# Autodesk Inventor assembly: marco
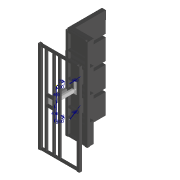
[picture p0: Inventor's stored thumbnail of the model, 180x180]
Saved by Autodesk Inventor 2021 (Build 250183000, 183)
## iProperties
Created: 2021-04-11
Part Number: marco
Document SubType Name: Assembly
Designer: equip
Mass: 525959 g
Surface Area: 133006 cm^2
Volume: 315655 cm^3
Density: 1.66625 g/cm^3
_SolveAssemblyDoc: Frame Generator Solve Assembly
_Version: 25.0.0
Author: equip
## Documents named in this file (12)
- C:\Users\Santiago Suárez\Documents\GitHub\Dis.-Mecatronico-E6\inventor proyecto\marco.iam
- C:\Users\Santiago Suárez\Documents\GitHub\Dis.-Mecatronico-E6\inventor proyecto\placa centro.ipt
- C:\Users\Santiago Suárez\Documents\GitHub\Dis.-Mecatronico-E6\inventor proyecto\Silla del marco.ipt
- C:\Users\Santiago Suárez\Documents\GitHub\Dis.-Mecatronico-E6\inventor proyecto\cilindro\cilindro.iam
- C:\Users\Santiago Suárez\Documents\GitHub\Dis.-Mecatronico-E6\inventor proyecto\marco inferior.ipt
- C:\Users\Santiago Suárez\Documents\GitHub\Dis.-Mecatronico-E6\inventor proyecto\marco\Frame\Marco Inferior.iam
- C:\Users\Santiago Suárez\Documents\GitHub\Dis.-Mecatronico-E6\inventor proyecto\MarcoSuperior.iam
- C:\Users\Santiago Suárez\Documents\GitHub\Dis.-Mecatronico-E6\inventor proyecto\Motor1.ipt
- C:\Users\Santiago Suárez\Documents\GitHub\Dis.-Mecatronico-E6\inventor proyecto\PlacaInferior.ipt
- C:\Users\Santiago Suárez\Documents\GitHub\Dis.-Mecatronico-E6\inventor proyecto\Eje.ipt
- C:\Users\Santiago Suárez\Documents\GitHub\Dis.-Mecatronico-E6\inventor proyecto\manivela.ipt
- C:\Users\Santiago Suárez\Documents\GitHub\Dis.-Mecatronico-E6\inventor proyecto\Biela.ipt
## Components (17 placed, 11 different names)
1. placa centro:1 — Rigid:3, Rigid:8
2. marco inferior:1
3. Marco Inferior:1 [sub-assembly] — Mate:23, Mate:24
4. MarcoSuperior:1 [sub-assembly] — Rigid:3, Mate:21, Mate:22, Ball:3, Ball:4
5. Motor1:1 — Rigid:5, Rotational:1, Rotational:2
6. PlacaInferior:1 — Mate:23, Mate:24, Mate:25, Mate:26, Mate:27, Rigid:5
7. cilindro:1 [sub-assembly] — Mate:25, Mate:26, Mate:27, Rigid:8
8. Eje:1 — Rotational:1, Rigid:7
9. Eje:2 — Rotational:2, Rigid:6
10. manivela:1 — Rigid:6, Ball:1
11. manivela:2 — Rigid:7, Ball:2
12. Biela:1 — Ball:1, Ball:3
13. Biela:2 — Ball:2, Ball:4
14. Silla del marco:1 — Mate:21, Mate:22
15. Silla del marco:2
16. Silla del marco:3
17. Silla del marco:4
## Component patterns: (4 elements, first: Silla del marco:1)
## Relationships (18: Mate 7, WeldJoint 5, BallJoint 4, RevoluteJoint 2)
- Rigid:3 [WeldJoint]: placa centro:1 ↔ MarcoSuperior:1
- Mate:21 (-10 mm): MarcoSuperior:1 ↔ Silla del marco:1
- Mate:22: MarcoSuperior:1 ↔ Silla del marco:1
- Mate:23: Marco Inferior:1 ↔ PlacaInferior:1
- Mate:24: Marco Inferior:1 ↔ PlacaInferior:1
- Mate:25: PlacaInferior:1 ↔ cilindro:1
- Mate:26 (88.5 mm): PlacaInferior:1 ↔ cilindro:1
- Mate:27 (-100 mm): PlacaInferior:1 ↔ cilindro:1
- Rigid:5 [WeldJoint]: Motor1:1 ↔ PlacaInferior:1
- Rotational:1 [RevoluteJoint]: Motor1:1 ↔ Eje:1
- Rotational:2 [RevoluteJoint]: Motor1:1 ↔ Eje:2
- Rigid:6 [WeldJoint]: Eje:2 ↔ manivela:1
- Rigid:7 [WeldJoint]: Eje:1 ↔ manivela:2
- Ball:1: manivela:1 ↔ Biela:1
- Ball:2: manivela:2 ↔ Biela:2
- Ball:3: MarcoSuperior:1 ↔ Biela:1
- Ball:4: MarcoSuperior:1 ↔ Biela:2
- Rigid:8 [WeldJoint]: placa centro:1 ↔ cilindro:1
## Named parameters: sa_0 = 470880, sa_1 = 470880, sa_2 = 470880, sa_3 = 470880, sa_4 = 1000, sa_5 = 1e+06, sa_6 = 1e+06
note: some values were not read from the file. Shown as the stored number, unit unknown: "sa_0", "sa_1", "sa_2", "sa_3", "sa_4", "sa_5", "sa_6".
